# Autodesk Inventor assembly: Клапан1
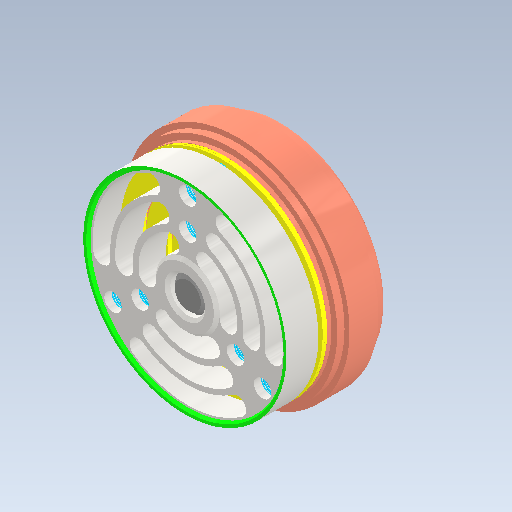
[picture p0: Inventor's stored thumbnail of the model, 512x512]
Saved by Autodesk Inventor 2021 (Build 250183000, 183)
## iProperties
Created: 2020-11-07
Part Number: Клапан1
Document SubType Name: Assembly
Designer: Тимоха
Author: Тимоха
## Documents named in this file (7)
- C:\Users\Тимоха\Desktop\КР Компрессор\compressor\Клапан1.iam
- C:\Users\Тимоха\Desktop\КР Компрессор\compressor\Клапан\Гайка М24-6H ГОСТ 5915-70.ipt
- C:\Users\Тимоха\Desktop\КР Компрессор\compressor\Клапан\Ограничитель .ipt
- C:\Users\Тимоха\Desktop\КР Компрессор\compressor\Клапан\Пластина.ipt
- C:\Users\Тимоха\Desktop\КР Компрессор\compressor\Клапан\Пружина_1.ipt
- C:\Users\Тимоха\Desktop\КР Компрессор\compressor\Клапан\Седло .ipt
- C:\Users\Тимоха\Desktop\КР Компрессор\compressor\Клапан\Шпилька М24-6gx48 ГОСТ 22038-76.ipt
## Components (12 placed, 6 different names)
1. Гайка М24-6H ГОСТ 5915-70:1 — Цилиндрический:1
2. Ограничитель :1 — С поворотом:3
3. Пластина:1 — Совмещение:1, Совмещение:2, Совмещение:3, Совмещение:4, Совмещение:5, Совмещение:6, С поворотом:1, С поворотом:4
4. Седло :1 — С поворотом:1, С поворотом:2
5. Шпилька М24-6gx48 ГОСТ 22038-76:1 — С поворотом:4, Цилиндрический:1
6. Ограничитель :2 — С поворотом:2, С поворотом:3
7. Пружина_1:1 — Совмещение:2
8. Пружина_1:2 — Совмещение:3
9. Пружина_1:3 — Совмещение:4
10. Пружина_1:4 — Совмещение:1
11. Пружина_1:5 — Совмещение:6
12. Пружина_1:6 — Совмещение:5
## Relationships (11: Mate 6, RevoluteJoint 4, CylindricalJoint 1)
- Совмещение:1 [Mate]: Пластина:1 ↔ Пружина_1:4
- Совмещение:2 [Mate]: Пластина:1 ↔ Пружина_1:1
- Совмещение:3 [Mate]: Пластина:1 ↔ Пружина_1:2
- Совмещение:4 [Mate]: Пластина:1 ↔ Пружина_1:3
- Совмещение:5 [Mate]: Пластина:1 ↔ Пружина_1:6
- Совмещение:6 [Mate]: Пластина:1 ↔ Пружина_1:5
- С поворотом:1 [RevoluteJoint]: Пластина:1 ↔ Седло :1
- С поворотом:2 [RevoluteJoint]: Седло :1 ↔ Ограничитель :2
- С поворотом:3 [RevoluteJoint]: Ограничитель :1 ↔ Ограничитель :2
- С поворотом:4 [RevoluteJoint]: Пластина:1 ↔ Шпилька М24-6gx48 ГОСТ 22038-76:1
- Цилиндрический:1 [CylindricalJoint]: Гайка М24-6H ГОСТ 5915-70:1 ↔ Шпилька М24-6gx48 ГОСТ 22038-76:1
